# Autodesk Inventor assembly: Planktoscope_Mini_Peristalticpump
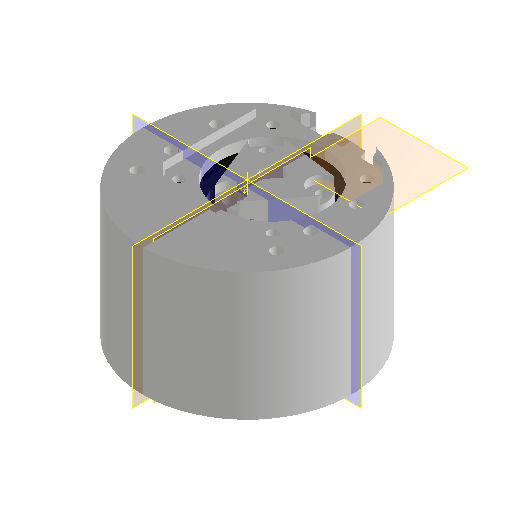
[picture p0: Inventor's stored thumbnail of the model, 512x512]
Saved by Autodesk Inventor 2022 (Build 260153000, 153)
## iProperties
Created: 2022-11-30
Part Number: Planktoscope_Mini_Peristalticpump
Document SubType Name: Assembly
Designer: diederichbenedict
Author: diederichbenedict
## Documents named in this file (6)
- C:\Users\diederichbenedict\Dropbox\Dokumente\Promotion\PROJECTS\Matchboxscope\INVENTOR\MATCHBOXSCOPE\Planktoscope_Mini_Peristalticpump.iam
- C:\Users\diederichbenedict\Dropbox\Dokumente\Promotion\PROJECTS\Matchboxscope\INVENTOR\MATCHBOXSCOPE\00_Stepper_Motor_28BYJ-48.ipt
- C:\Users\diederichbenedict\Dropbox\Dokumente\Promotion\PROJECTS\Matchboxscope\INVENTOR\MATCHBOXSCOPE\Matchboxscope_bottom_v0.ipt
- C:\Users\diederichbenedict\Dropbox\Dokumente\Promotion\PROJECTS\Matchboxscope\INVENTOR\MATCHBOXSCOPE\Pump_Rotation.ipt
- C:\Users\diederichbenedict\Dropbox\Dokumente\Promotion\PROJECTS\Matchboxscope\INVENTOR\MATCHBOXSCOPE\Pump_Base_Motor.ipt
- C:\Users\diederichbenedict\Dropbox\Dokumente\Promotion\PROJECTS\Matchboxscope\INVENTOR\MATCHBOXSCOPE\Pump_Lid.ipt
## Components (5 placed, 5 different names)
1. Pump_Base_Motor:1 — Passend:1, Winkel:1, Winkel:2, Einfügen:3, Passend:7
2. Pump_Lid:1
3. Pump_Rotation:1 — Einfügen:3
4. 00_Stepper_Motor_28BYJ-48:1 — Passend:1, Winkel:1, Winkel:2, Passend:2, Passend:3
5. Matchboxscope_bottom_v0:1 — Passend:2, Passend:3
## Relationships (7: Mate 4, Angle 2, Insert 1)
- Passend:1 [Mate]: Pump_Base_Motor:1 ↔ 00_Stepper_Motor_28BYJ-48:1
- Winkel:1 [Angle] (0.06 deg): Pump_Base_Motor:1 ↔ 00_Stepper_Motor_28BYJ-48:1
- Winkel:2 [Angle] (0.06 deg): Pump_Base_Motor:1 ↔ 00_Stepper_Motor_28BYJ-48:1
- Passend:2 [Mate]: 00_Stepper_Motor_28BYJ-48:1 ↔ Matchboxscope_bottom_v0:1
- Passend:3 [Mate] (20 mm): 00_Stepper_Motor_28BYJ-48:1 ↔ Matchboxscope_bottom_v0:1
- Einfügen:3 [Insert]: Pump_Base_Motor:1 ↔ Pump_Rotation:1
- Passend:7 [Mate]: Pump_Base_Motor:1
